# Autodesk Inventor assembly: Full assembly
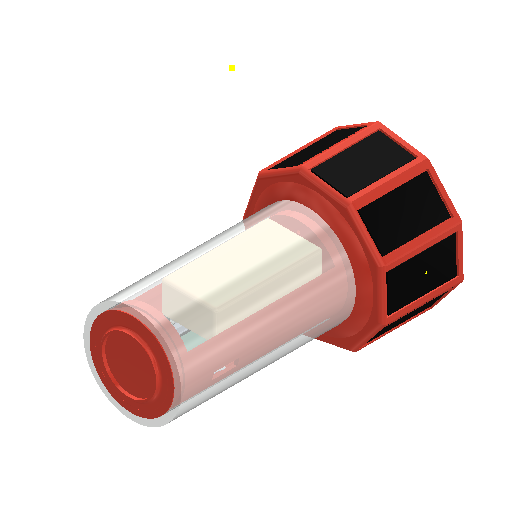
[picture p0: Inventor's stored thumbnail of the model, 512x512]
Saved by Autodesk Inventor 2025 (Build 290162000, 162)
## iProperties
Created: 2025-04-17
Part Number: Full assembly
Document SubType Name: Assembly
Designer: MK92
Sending System: Autodesk Translation Framework v14.4.0.0
Preprocessor: ST-DEVELOPER v20.1
Title: Full assembly.step
## Documents named in this file (7)
- C:\Users\MK92\OneDrive - University of South Carolina\Github Repos\UAV-Deployable-Stage-Height-Sensor\system_design\Georgetown\V0.5\CAD\CAD V 0.5.2\Full assembly 2.iam
- C:\Users\MK92\OneDrive - University of South Carolina\Github Repos\UAV-Deployable-Stage-Height-Sensor\system_design\Georgetown\V0.5\CAD\CAD V 0.5.2\PCB tray CAD v2.ipt
- C:\Users\MK92\OneDrive - University of South Carolina\Github Repos\UAV-Deployable-Stage-Height-Sensor\system_design\Georgetown\V0.5\CAD\CAD V 0.5.2\Clear Tube v19.iam
- C:\Users\MK92\OneDrive - University of South Carolina\Github Repos\UAV-Deployable-Stage-Height-Sensor\system_design\Georgetown\V0.5\CAD\CAD V 0.5.2\Battery.ipt
- C:\Users\MK92\OneDrive - University of South Carolina\Github Repos\UAV-Deployable-Stage-Height-Sensor\system_design\Georgetown\V0.5\CAD\CAD V 0.5.2\Ultrasonic HCSR04.ipt
- C:\Users\MK92\OneDrive - University of South Carolina\Github Repos\UAV-Deployable-Stage-Height-Sensor\system_design\Georgetown\V0.5\CAD\CAD V 0.5.2\Solar Panel.ipt
- C:\Users\MK92\OneDrive - University of South Carolina\Github Repos\UAV-Deployable-Stage-Height-Sensor\system_design\Georgetown\V0.5\CAD\CAD V 0.5.2\Main Board\main_board\main_board.iam
## Components (14 placed, 6 different names)
1. PCB tray CAD v2:1 — Mate:1, Mate:2, Mate:3, Mate:4, Rigid:1, Flush:1
2. Clear Tube v19:1 [sub-assembly]
3. Battery:1
4. Ultrasonic HCSR04:1
5. main_board:1 [sub-assembly] — Flush:1
6. Solar Panel:1 — Mate:1, Mate:2, Mate:3, Mate:4, Rigid:1
7. Solar Panel:2
8. Solar Panel:3
9. Solar Panel:4
10. Solar Panel:5
11. Solar Panel:6
12. Solar Panel:7
13. Solar Panel:8
14. Solar Panel:9
## Component patterns: (9 elements, first: Solar Panel:1)
## Relationships (6: Mate 4, WeldJoint 1, Flush 1)
- Mate:1: PCB tray CAD v2:1 ↔ Solar Panel:1
- Mate:2 (7.051 mm): PCB tray CAD v2:1 ↔ Solar Panel:1
- Mate:3: PCB tray CAD v2:1 ↔ Solar Panel:1
- Mate:4: PCB tray CAD v2:1 ↔ Solar Panel:1
- Rigid:1 [WeldJoint]: PCB tray CAD v2:1 ↔ Solar Panel:1
- Flush:1: PCB tray CAD v2:1 ↔ main_board:1
